# Autodesk Inventor assembly: Wrist Axis 4 Assembly
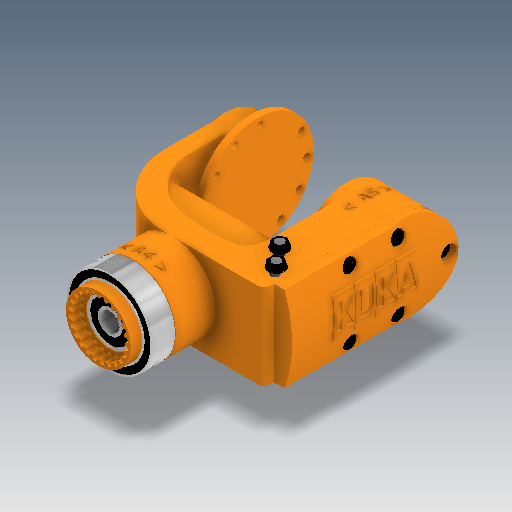
[picture p0: Inventor's stored thumbnail of the model, 512x512]
Saved by Autodesk Inventor 2020 (Build 240168000, 168)
## iProperties
Created: 2021-07-18
Part Number: Wrist Axis 4 Assembly
Document SubType Name: Assembly
Designer: Coy
Author: Coy
## Documents named in this file (19)
- E:\Documents\3D Files\Project 3D Models\Industrial 6 Axis Robot Arm\4th 5th amd 6th axis model\V2\Assemblys\KR500 Wrist Axis 4 Assembly.iam
- E:\Documents\3D Files\Project 3D Models\Industrial 6 Axis Robot Arm\4th 5th amd 6th axis model\V2\Wrist Axis 4 Frame.ipt
- E:\Documents\3D Files\Project 3D Models\Industrial 6 Axis Robot Arm\4th 5th amd 6th axis model\V2\Bearings\40mm ID 52mm OD 7mm Deep Roller Bearing.ipt
- E:\Documents\3D Files\Project 3D Models\Industrial 6 Axis Robot Arm\4th 5th amd 6th axis model\V2\Bearings\12mm ID 28mm OD 8mm Deep Roller Bearing.ipt
- E:\Documents\3D Files\Project 3D Models\Industrial 6 Axis Robot Arm\4th 5th amd 6th axis model\V2\Bearings\5mm ID 8mm OD 2.5mm Deep Roller Bearing.ipt
- E:\Documents\3D Files\Project 3D Models\Industrial 6 Axis Robot Arm\4th 5th amd 6th axis model\V2\M12 Hollow Shaft With 12mm Chamfered Male Fitting.ipt
- E:\Documents\3D Files\Project 3D Models\Industrial 6 Axis Robot Arm\4th 5th amd 6th axis model\V2\Gears and Couplers\M5 36 Tooth D Profile GT2 Pully.ipt
- E:\Documents\3D Files\Project 3D Models\Industrial 6 Axis Robot Arm\4th 5th amd 6th axis model\V2\Gears and Couplers\M10 36 Tooth GT2 Pully.ipt
- E:\Documents\3D Files\Project 3D Models\Industrial 6 Axis Robot Arm\4th 5th amd 6th axis model\V2\Shafts and Rods\M5 60mm Threaded Rod.ipt
- E:\Documents\3D Files\Project 3D Models\Industrial 6 Axis Robot Arm\4th 5th amd 6th axis model\V2\M5 Chamfered Belt Guide .ipt
- E:\Documents\3D Files\Project 3D Models\Industrial 6 Axis Robot Arm\4th 5th amd 6th axis model\V2\M5 GT2 Idler Pulley.ipt
- E:\Documents\3D Files\Project 3D Models\Industrial 6 Axis Robot Arm\4th 5th amd 6th axis model\V2\Nuts and Bolts\M5 Nut.ipt
- E:\Documents\3D Files\Project 3D Models\Industrial 6 Axis Robot Arm\4th 5th amd 6th axis model\V2\Nuts and Bolts\M5 Washer.ipt
- E:\Documents\3D Files\Project 3D Models\Industrial 6 Axis Robot Arm\4th 5th amd 6th axis model\V2\Nuts and Bolts\M5 7mm OD 8mm Deep Threaded Insert.ipt
- E:\Documents\3D Files\Project 3D Models\Industrial 6 Axis Robot Arm\4th 5th amd 6th axis model\V2\Wrist Axis 5 Mounting Plate.ipt
- E:\Documents\3D Files\Project 3D Models\Industrial 6 Axis Robot Arm\4th 5th amd 6th axis model\V2\Nuts and Bolts\M5 x 12 Socket Head Bolt.ipt
- E:\Documents\3D Files\Project 3D Models\Industrial 6 Axis Robot Arm\4th 5th amd 6th axis model\V2\Wrist Main Plate Cover Bearing Insert.ipt
- E:\Documents\3D Files\Project 3D Models\Industrial 6 Axis Robot Arm\4th 5th amd 6th axis model\V2\Shafts and Rods\M5 D Profile Rotary Shaft 50mm.ipt
- E:\Documents\3D Files\Project 3D Models\Industrial 6 Axis Robot Arm\4th 5th amd 6th axis model\V2\Wrist Main Plate Cover Main.ipt
## Components (56 placed, 18 different names)
1. Wrist Axis 4 Frame:1 — Mate:1, Flush:1, Mate:2, Flush:2, Mate:3, Flush:3, Mate:4, Flush:4, Mate:5, Mate:6, Tangent:1, Flush:16, Tangent:2, Flush:17, Mate:24, Mate:25, Mate:46, Mate:47, Mate:48, Mate:49, Mate:66, Flush:20, Mate:67, Flush:21, Mate:68, Flush:22, Mate:69, Flush:23, Mate:70, Flush:24, Mate:76, Mate:77, Mate:79, Flush:25, Mate:100, Mate:101, Mate:102, Mate:103, Mate:104, Mate:105
2. 40mm ID 52mm OD 7mm Deep Roller Bearing:1 — Mate:5, Mate:6, Mate:78
3. 12mm ID 28mm OD 8mm Deep Roller Bearing:1 — Mate:4, Flush:4, Mate:75
4. 12mm ID 28mm OD 8mm Deep Roller Bearing:2 — Mate:3, Flush:3, Mate:11, Flush:9
5. 12mm ID 28mm OD 8mm Deep Roller Bearing:3 — Mate:1, Flush:1
6. 12mm ID 28mm OD 8mm Deep Roller Bearing:4 — Mate:2, Flush:2
7. 5mm ID 8mm OD 2.5mm Deep Roller Bearing:3 — Mate:13, Flush:11, Mate:107
8. 5mm ID 8mm OD 2.5mm Deep Roller Bearing:4 — Mate:12, Flush:10
9. M12 Hollow Shaft With 12mm Chamfered Male Fitting:1 — Mate:11, Flush:9, Mate:12, Flush:10, Mate:13, Flush:11, Mate:18, Flush:14, Rotation:3, Mate:73
10. M5 36 Tooth D Profile GT2 Pully:2 — Mate:108, Mate:109, Rotation:4
11. M10 36 Tooth GT2 Pully:2 — Mate:18, Flush:14, Rotation:3, Mate:109
12. M5 60mm Threaded Rod:1 — Tangent:1, Flush:16, Mate:20, Mate:21, Mate:26, Mate:28, Mate:34, Mate:36, Mate:42, Mate:44, Mate:50, Mate:52, Mate:54, Mate:56
13. M5 60mm Threaded Rod:2 — Tangent:2, Flush:17, Mate:22, Mate:23, Mate:27, Mate:29, Mate:35, Mate:37, Mate:43, Mate:45, Mate:51, Mate:53, Mate:55, Mate:57
14. M5 Chamfered Belt Guide :1 — Mate:28, Mate:31
15. M5 Chamfered Belt Guide :2 — Mate:29, Mate:30
16. M5 Chamfered Belt Guide :3 — Mate:37, Mate:41
17. M5 Chamfered Belt Guide :4 — Mate:36, Mate:40
18. M5 Chamfered Belt Guide :5 — Mate:27, Mate:33, Mate:61
19. M5 Chamfered Belt Guide :6 — Mate:35, Mate:39, Mate:59
20. M5 Chamfered Belt Guide :7 — Mate:26, Mate:32, Mate:60
21. M5 Chamfered Belt Guide :8 — Mate:34, Mate:38, Mate:58
22. M5 GT2 Idler Pulley:1 — Mate:20, Mate:24, Flush:18, Mate:31, Mate:38
23. M5 GT2 Idler Pulley:2 — Mate:21, Mate:25, Flush:19, Mate:32, Mate:40
24. M5 GT2 Idler Pulley:3 — Mate:22, Flush:18, Mate:30, Mate:39
25. M5 GT2 Idler Pulley:4 — Mate:23, Flush:19, Mate:33, Mate:41
26. M5 Nut:1 — Mate:56, Mate:58
27. M5 Nut:2 — Mate:57, Mate:59
28. M5 Nut:3 — Mate:55, Mate:61
29. M5 Nut:4 — Mate:54, Mate:60
30. M5 Nut:5 — Mate:53, Mate:65
31. M5 Nut:6 — Mate:52, Mate:64
32. M5 Nut:7 — Mate:50, Mate:62
33. M5 Nut:8 — Mate:51, Mate:63
34. M5 Washer:1 — Mate:42, Mate:46, Mate:64
35. M5 Washer:2 — Mate:43, Mate:47, Mate:65
36. M5 Washer:3 — Mate:44, Mate:48, Mate:62
37. M5 Washer:4 — Mate:45, Mate:49, Mate:63
38. M5 7mm OD 8mm Deep Threaded Insert:1 — Mate:69, Flush:23, Mate:95
39. M5 7mm OD 8mm Deep Threaded Insert:2 — Mate:66, Flush:20, Mate:98
40. M5 7mm OD 8mm Deep Threaded Insert:3 — Mate:68, Flush:22, Mate:96
41. M5 7mm OD 8mm Deep Threaded Insert:4 — Mate:67, Flush:21, Mate:97
42. M5 7mm OD 8mm Deep Threaded Insert:5 — Mate:70, Flush:24, Mate:99
43. M5 Washer:5 — Mate:74
44. M5 Washer:6 — Mate:73, Mate:74
45. Wrist Axis 5 Mounting Plate:1 — Mate:75, Mate:76
46. 40mm ID 52mm OD 7mm Deep Roller Bearing:2 — Mate:77, Mate:78
47. 5mm ID 8mm OD 2.5mm Deep Roller Bearing:5 — Mate:79, Flush:25
48. M5 x 12 Socket Head Bolt:1 — Mate:93, Mate:99, Mate:100, Mate:110
49. M5 x 12 Socket Head Bolt:2 — Mate:95, Mate:101
50. M5 x 12 Socket Head Bolt:3 — Mate:94, Mate:97, Mate:103, Mate:111
51. M5 x 12 Socket Head Bolt:4 — Mate:98, Mate:104
52. M5 x 12 Socket Head Bolt:5 — Mate:96, Mate:102
53. Wrist Main Plate Cover Bearing Insert:1 — Mate:93, Mate:94, Mate:105, Mate:106, Flush:26, Flush:27, Mate:112
54. 5mm ID 8mm OD 2.5mm Deep Roller Bearing:6 — Mate:106, Flush:26
55. M5 D Profile Rotary Shaft 50mm:1 — Mate:107, Mate:108, Rotation:4, Flush:27
56. Wrist Main Plate Cover Main:1 — Mate:110, Mate:111, Mate:112
## Relationships (112: Mate 88, Flush 20, RelateRotation 2, Tangent 2)
- Mate:1: Wrist Axis 4 Frame:1 ↔ 12mm ID 28mm OD 8mm Deep Roller Bearing:3
- Flush:1: Wrist Axis 4 Frame:1 ↔ 12mm ID 28mm OD 8mm Deep Roller Bearing:3
- Mate:2: Wrist Axis 4 Frame:1 ↔ 12mm ID 28mm OD 8mm Deep Roller Bearing:4
- Flush:2: Wrist Axis 4 Frame:1 ↔ 12mm ID 28mm OD 8mm Deep Roller Bearing:4
- Mate:3: Wrist Axis 4 Frame:1 ↔ 12mm ID 28mm OD 8mm Deep Roller Bearing:2
- Flush:3: Wrist Axis 4 Frame:1 ↔ 12mm ID 28mm OD 8mm Deep Roller Bearing:2
- Mate:4: Wrist Axis 4 Frame:1 ↔ 12mm ID 28mm OD 8mm Deep Roller Bearing:1
- Flush:4: Wrist Axis 4 Frame:1 ↔ 12mm ID 28mm OD 8mm Deep Roller Bearing:1
- Mate:5: Wrist Axis 4 Frame:1 ↔ 40mm ID 52mm OD 7mm Deep Roller Bearing:1
- Mate:6 (0.5 mm): Wrist Axis 4 Frame:1 ↔ 40mm ID 52mm OD 7mm Deep Roller Bearing:1
- Mate:11: 12mm ID 28mm OD 8mm Deep Roller Bearing:2 ↔ M12 Hollow Shaft With 12mm Chamfered Male Fitting:1
- Flush:9 (-10.75 mm): 12mm ID 28mm OD 8mm Deep Roller Bearing:2 ↔ M12 Hollow Shaft With 12mm Chamfered Male Fitting:1
- Mate:12: 5mm ID 8mm OD 2.5mm Deep Roller Bearing:4 ↔ M12 Hollow Shaft With 12mm Chamfered Male Fitting:1
- Flush:10: 5mm ID 8mm OD 2.5mm Deep Roller Bearing:4 ↔ M12 Hollow Shaft With 12mm Chamfered Male Fitting:1
- Mate:13: 5mm ID 8mm OD 2.5mm Deep Roller Bearing:3 ↔ M12 Hollow Shaft With 12mm Chamfered Male Fitting:1
- Flush:11: 5mm ID 8mm OD 2.5mm Deep Roller Bearing:3 ↔ M12 Hollow Shaft With 12mm Chamfered Male Fitting:1
- Mate:18: M12 Hollow Shaft With 12mm Chamfered Male Fitting:1 ↔ M10 36 Tooth GT2 Pully:2
- Flush:14: M12 Hollow Shaft With 12mm Chamfered Male Fitting:1 ↔ M10 36 Tooth GT2 Pully:2
- Rotation:3 [RelateRotation] (1 ul): M12 Hollow Shaft With 12mm Chamfered Male Fitting:1 ↔ M10 36 Tooth GT2 Pully:2
- Tangent:1 (0.1 mm): Wrist Axis 4 Frame:1 ↔ M5 60mm Threaded Rod:1
- Flush:16 (-4 mm): Wrist Axis 4 Frame:1 ↔ M5 60mm Threaded Rod:1
- Tangent:2 (0.1 mm): Wrist Axis 4 Frame:1 ↔ M5 60mm Threaded Rod:2
- Flush:17 (-4 mm): Wrist Axis 4 Frame:1 ↔ M5 60mm Threaded Rod:2
- Mate:20: M5 60mm Threaded Rod:1 ↔ M5 GT2 Idler Pulley:1
- Mate:21: M5 60mm Threaded Rod:1 ↔ M5 GT2 Idler Pulley:2
- Mate:22: M5 60mm Threaded Rod:2 ↔ M5 GT2 Idler Pulley:3
- Mate:23: M5 60mm Threaded Rod:2 ↔ M5 GT2 Idler Pulley:4
- Mate:24 (10 mm): Wrist Axis 4 Frame:1 ↔ M5 GT2 Idler Pulley:1
- Flush:18: M5 GT2 Idler Pulley:1 ↔ M5 GT2 Idler Pulley:3
- Mate:25 (10 mm): Wrist Axis 4 Frame:1 ↔ M5 GT2 Idler Pulley:2
- Flush:19: M5 GT2 Idler Pulley:2 ↔ M5 GT2 Idler Pulley:4
- Mate:26: M5 60mm Threaded Rod:1 ↔ M5 Chamfered Belt Guide :7
- Mate:27: M5 60mm Threaded Rod:2 ↔ M5 Chamfered Belt Guide :5
- Mate:28: M5 60mm Threaded Rod:1 ↔ M5 Chamfered Belt Guide :1
- Mate:29: M5 60mm Threaded Rod:2 ↔ M5 Chamfered Belt Guide :2
- Mate:30 (0.2 mm): M5 Chamfered Belt Guide :2 ↔ M5 GT2 Idler Pulley:3
- Mate:31 (0.2 mm): M5 Chamfered Belt Guide :1 ↔ M5 GT2 Idler Pulley:1
- Mate:32 (0.2 mm): M5 Chamfered Belt Guide :7 ↔ M5 GT2 Idler Pulley:2
- Mate:33 (0.2 mm): M5 Chamfered Belt Guide :5 ↔ M5 GT2 Idler Pulley:4
- Mate:34: M5 60mm Threaded Rod:1 ↔ M5 Chamfered Belt Guide :8
- Mate:35: M5 60mm Threaded Rod:2 ↔ M5 Chamfered Belt Guide :6
- Mate:36: M5 60mm Threaded Rod:1 ↔ M5 Chamfered Belt Guide :4
- Mate:37: M5 60mm Threaded Rod:2 ↔ M5 Chamfered Belt Guide :3
- Mate:38 (0.2 mm): M5 Chamfered Belt Guide :8 ↔ M5 GT2 Idler Pulley:1
- Mate:39: M5 Chamfered Belt Guide :6 ↔ M5 GT2 Idler Pulley:3
- Mate:40 (0.2 mm): M5 Chamfered Belt Guide :4 ↔ M5 GT2 Idler Pulley:2
- Mate:41: M5 Chamfered Belt Guide :3 ↔ M5 GT2 Idler Pulley:4
- Mate:42: M5 60mm Threaded Rod:1 ↔ M5 Washer:1
- Mate:43: M5 60mm Threaded Rod:2 ↔ M5 Washer:2
- Mate:44: M5 60mm Threaded Rod:1 ↔ M5 Washer:3
- Mate:45: M5 60mm Threaded Rod:2 ↔ M5 Washer:4
- Mate:46: Wrist Axis 4 Frame:1 ↔ M5 Washer:1
- Mate:47: Wrist Axis 4 Frame:1 ↔ M5 Washer:2
- Mate:48: Wrist Axis 4 Frame:1 ↔ M5 Washer:3
- Mate:49: Wrist Axis 4 Frame:1 ↔ M5 Washer:4
- Mate:50: M5 60mm Threaded Rod:1 ↔ M5 Nut:7
- Mate:51: M5 60mm Threaded Rod:2 ↔ M5 Nut:8
- Mate:52: M5 60mm Threaded Rod:1 ↔ M5 Nut:6
- Mate:53: M5 60mm Threaded Rod:2 ↔ M5 Nut:5
- Mate:54: M5 60mm Threaded Rod:1 ↔ M5 Nut:4
- Mate:55: M5 60mm Threaded Rod:2 ↔ M5 Nut:3
- Mate:56: M5 60mm Threaded Rod:1 ↔ M5 Nut:1
- Mate:57: M5 60mm Threaded Rod:2 ↔ M5 Nut:2
- Mate:58: M5 Chamfered Belt Guide :8 ↔ M5 Nut:1
- Mate:59: M5 Chamfered Belt Guide :6 ↔ M5 Nut:2
- Mate:60: M5 Chamfered Belt Guide :7 ↔ M5 Nut:4
- Mate:61: M5 Chamfered Belt Guide :5 ↔ M5 Nut:3
- Mate:62: M5 Nut:7 ↔ M5 Washer:3
- Mate:63: M5 Nut:8 ↔ M5 Washer:4
- Mate:64: M5 Nut:6 ↔ M5 Washer:1
- Mate:65: M5 Nut:5 ↔ M5 Washer:2
- Mate:66: Wrist Axis 4 Frame:1 ↔ M5 7mm OD 8mm Deep Threaded Insert:2
- Flush:20: Wrist Axis 4 Frame:1 ↔ M5 7mm OD 8mm Deep Threaded Insert:2
- Mate:67: Wrist Axis 4 Frame:1 ↔ M5 7mm OD 8mm Deep Threaded Insert:4
- Flush:21: Wrist Axis 4 Frame:1 ↔ M5 7mm OD 8mm Deep Threaded Insert:4
- Mate:68: Wrist Axis 4 Frame:1 ↔ M5 7mm OD 8mm Deep Threaded Insert:3
- Flush:22: Wrist Axis 4 Frame:1 ↔ M5 7mm OD 8mm Deep Threaded Insert:3
- Mate:69: Wrist Axis 4 Frame:1 ↔ M5 7mm OD 8mm Deep Threaded Insert:1
- Flush:23: Wrist Axis 4 Frame:1 ↔ M5 7mm OD 8mm Deep Threaded Insert:1
- Mate:70: Wrist Axis 4 Frame:1 ↔ M5 7mm OD 8mm Deep Threaded Insert:5
- Flush:24: Wrist Axis 4 Frame:1 ↔ M5 7mm OD 8mm Deep Threaded Insert:5
- Mate:73: M12 Hollow Shaft With 12mm Chamfered Male Fitting:1 ↔ M5 Washer:6
- Mate:74: M5 Washer:5 ↔ M5 Washer:6
- Mate:75: 12mm ID 28mm OD 8mm Deep Roller Bearing:1 ↔ Wrist Axis 5 Mounting Plate:1
- Mate:76 (0.5 mm): Wrist Axis 4 Frame:1 ↔ Wrist Axis 5 Mounting Plate:1
- Mate:77: Wrist Axis 4 Frame:1 ↔ 40mm ID 52mm OD 7mm Deep Roller Bearing:2
- Mate:78: 40mm ID 52mm OD 7mm Deep Roller Bearing:1 ↔ 40mm ID 52mm OD 7mm Deep Roller Bearing:2
- Mate:79: Wrist Axis 4 Frame:1 ↔ 5mm ID 8mm OD 2.5mm Deep Roller Bearing:5
- Flush:25: Wrist Axis 4 Frame:1 ↔ 5mm ID 8mm OD 2.5mm Deep Roller Bearing:5
- Mate:93: M5 x 12 Socket Head Bolt:1 ↔ Wrist Main Plate Cover Bearing Insert:1
- Mate:94: M5 x 12 Socket Head Bolt:3 ↔ Wrist Main Plate Cover Bearing Insert:1
- Mate:95: M5 7mm OD 8mm Deep Threaded Insert:1 ↔ M5 x 12 Socket Head Bolt:2
- Mate:96: M5 7mm OD 8mm Deep Threaded Insert:3 ↔ M5 x 12 Socket Head Bolt:5
- Mate:97: M5 7mm OD 8mm Deep Threaded Insert:4 ↔ M5 x 12 Socket Head Bolt:3
- Mate:98: M5 7mm OD 8mm Deep Threaded Insert:2 ↔ M5 x 12 Socket Head Bolt:4
- Mate:99: M5 7mm OD 8mm Deep Threaded Insert:5 ↔ M5 x 12 Socket Head Bolt:1
- Mate:100 (0.75 mm): Wrist Axis 4 Frame:1 ↔ M5 x 12 Socket Head Bolt:1
- Mate:101 (0.75 mm): Wrist Axis 4 Frame:1 ↔ M5 x 12 Socket Head Bolt:2
- Mate:102 (0.75 mm): Wrist Axis 4 Frame:1 ↔ M5 x 12 Socket Head Bolt:5
- Mate:103 (0.75 mm): Wrist Axis 4 Frame:1 ↔ M5 x 12 Socket Head Bolt:3
- Mate:104 (0.75 mm): Wrist Axis 4 Frame:1 ↔ M5 x 12 Socket Head Bolt:4
- Mate:105 (0.05 mm): Wrist Axis 4 Frame:1 ↔ Wrist Main Plate Cover Bearing Insert:1
- Mate:106: Wrist Main Plate Cover Bearing Insert:1 ↔ 5mm ID 8mm OD 2.5mm Deep Roller Bearing:6
- Flush:26: Wrist Main Plate Cover Bearing Insert:1 ↔ 5mm ID 8mm OD 2.5mm Deep Roller Bearing:6
- Mate:107: 5mm ID 8mm OD 2.5mm Deep Roller Bearing:3 ↔ M5 D Profile Rotary Shaft 50mm:1
- Mate:108: M5 36 Tooth D Profile GT2 Pully:2 ↔ M5 D Profile Rotary Shaft 50mm:1
- Mate:109 (0.15 mm): M5 36 Tooth D Profile GT2 Pully:2 ↔ M10 36 Tooth GT2 Pully:2
- Rotation:4 [RelateRotation] (5 ul): M5 36 Tooth D Profile GT2 Pully:2 ↔ M5 D Profile Rotary Shaft 50mm:1
- Flush:27 (-0.75 mm): Wrist Main Plate Cover Bearing Insert:1 ↔ M5 D Profile Rotary Shaft 50mm:1
- Mate:110: M5 x 12 Socket Head Bolt:1 ↔ Wrist Main Plate Cover Main:1
- Mate:111: M5 x 12 Socket Head Bolt:3 ↔ Wrist Main Plate Cover Main:1
- Mate:112 (0.05 mm): Wrist Main Plate Cover Bearing Insert:1 ↔ Wrist Main Plate Cover Main:1
